# Autodesk Inventor assembly: Planktoscope_Mini_v0
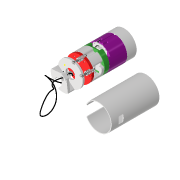
[picture p0: Inventor's stored thumbnail of the model, 180x180]
Saved by Autodesk Inventor 2022 (Build 260153000, 153)
## iProperties
Created: 2022-04-02
Part Number: Planktoscope_Mini_v0
Document SubType Name: Assembly
Designer: Prakash Lab
Author: Prakash Lab
## Documents named in this file (14)
- C:\Users\diederichbenedict\Dropbox\Dokumente\Promotion\PROJECTS\Matchboxscope\INVENTOR\MATCHBOXSCOPE\Planktoscope_Mini_v0.iam
- C:\Users\diederichbenedict\Dropbox\Dokumente\Promotion\PROJECTS\Matchboxscope\INVENTOR\MATCHBOXSCOPE\Matchboxscope_bottom_v0.ipt
- C:\Users\diederichbenedict\Dropbox\Dokumente\Promotion\PROJECTS\Matchboxscope\INVENTOR\MATCHBOXSCOPE\00_ESP3-CAM.iam
- C:\Users\diederichbenedict\Dropbox\Dokumente\Promotion\PROJECTS\Matchboxscope\INVENTOR\MATCHBOXSCOPE\00_Powerbank.ipt
- C:\Users\diederichbenedict\Dropbox\Dokumente\Promotion\PROJECTS\Matchboxscope\INVENTOR\MATCHBOXSCOPE\00_spring.ipt
- C:\Users\diederichbenedict\Documents\Inventor\Content Center Files\R2022\de-DE\DIN 912\DIN 912 - M3 x 0.5 x 25 x 18.ipt
- C:\Users\diederichbenedict\Dropbox\Dokumente\Promotion\PROJECTS\Matchboxscope\INVENTOR\MATCHBOXSCOPE\Matchboxscope_middle2_v2.ipt
- C:\Users\diederichbenedict\Dropbox\Dokumente\Promotion\PROJECTS\Matchboxscope\INVENTOR\MATCHBOXSCOPE\Anglerfish_Cameraspacer.ipt
- C:\Users\diederichbenedict\Dropbox\Dokumente\Promotion\PROJECTS\Matchboxscope\INVENTOR\MATCHBOXSCOPE\Matchboxscope_sample_universal_toslink.ipt
- C:\Users\diederichbenedict\Dropbox\Dokumente\Promotion\PROJECTS\Matchboxscope\INVENTOR\MATCHBOXSCOPE\Planktoscope_Mini_Peristalticpump.iam
- C:\Users\diederichbenedict\Dropbox\Dokumente\Promotion\PROJECTS\Matchboxscope\INVENTOR\MATCHBOXSCOPE\00_Toslink.ipt
- C:\Users\diederichbenedict\Dropbox\Dokumente\Promotion\PROJECTS\Matchboxscope\INVENTOR\MATCHBOXSCOPE\Planktoscope_Mini_Electronicbase.iam
- C:\Users\diederichbenedict\Dropbox\Dokumente\Promotion\PROJECTS\Matchboxscope\INVENTOR\MATCHBOXSCOPE\Planktoscope_connectortube.ipt
- C:\Users\diederichbenedict\Dropbox\Dokumente\Promotion\PROJECTS\Matchboxscope\INVENTOR\MATCHBOXSCOPE\Matchboxscope_layer_ikealamp.ipt
## Components (21 placed, 13 different names)
1. Matchboxscope_bottom_v0:1 — Mate:1, Mate:2, Mate:3, Mate:4, Flush:1, Einfügen:1, Winkel:1
2. 00_ESP3-CAM:1 [sub-assembly] — Mate:4, Flush:1, Passend:5
3. 00_Powerbank:1
4. 00_spring:1
5. DIN 912 - ersetzt durch DIN EN ISO 4762 M3 x 25:1 — Passend:6
6. DIN 912 - ersetzt durch DIN EN ISO 4762 M3 x 25:2
7. DIN 912 - ersetzt durch DIN EN ISO 4762 M3 x 25:3
8. 00_spring:3
9. 00_spring:4
10. DIN 912 - ersetzt durch DIN EN ISO 4762 M3 x 25:4
11. DIN 912 - ersetzt durch DIN EN ISO 4762 M3 x 25:5
12. DIN 912 - ersetzt durch DIN EN ISO 4762 M3 x 25:6
13. DIN 912 - ersetzt durch DIN EN ISO 4762 M3 x 25:7
14. Matchboxscope_middle2_v2:1 — Einfügen:1, Passend:5, Winkel:1, Passend:7
15. Anglerfish_Cameraspacer:1
16. Matchboxscope_sample_universal_toslink:1 — Passend:6, Passend:7, Einfügen:2
17. 00_Toslink:1 — Einfügen:2
18. Matchboxscope_layer_ikealamp:1
19. Planktoscope_Mini_Peristalticpump:1 [sub-assembly]
20. Planktoscope_Mini_Electronicbase:1 [sub-assembly]
21. Planktoscope_connectortube:1
## Relationships (11: Mate 7, Insert 2, Flush 1, Angle 1)
- Mate:1: Matchboxscope_bottom_v0:1
- Mate:2: Matchboxscope_bottom_v0:1
- Mate:3: Matchboxscope_bottom_v0:1
- Mate:4: Matchboxscope_bottom_v0:1 ↔ 00_ESP3-CAM:1
- Flush:1: Matchboxscope_bottom_v0:1 ↔ 00_ESP3-CAM:1
- Einfügen:1 [Insert]: Matchboxscope_bottom_v0:1 ↔ Matchboxscope_middle2_v2:1
- Passend:5 [Mate] (3 mm): 00_ESP3-CAM:1 ↔ Matchboxscope_middle2_v2:1
- Winkel:1 [Angle] (180 deg): Matchboxscope_bottom_v0:1 ↔ Matchboxscope_middle2_v2:1
- Passend:6 [Mate]: DIN 912 - ersetzt durch DIN EN ISO 4762 M3 x 25:1 ↔ Matchboxscope_sample_universal_toslink:1
- Passend:7 [Mate]: Matchboxscope_middle2_v2:1 ↔ Matchboxscope_sample_universal_toslink:1
- Einfügen:2 [Insert] (12 mm): Matchboxscope_sample_universal_toslink:1 ↔ 00_Toslink:1
